# Autodesk Inventor assembly: Scrambler II
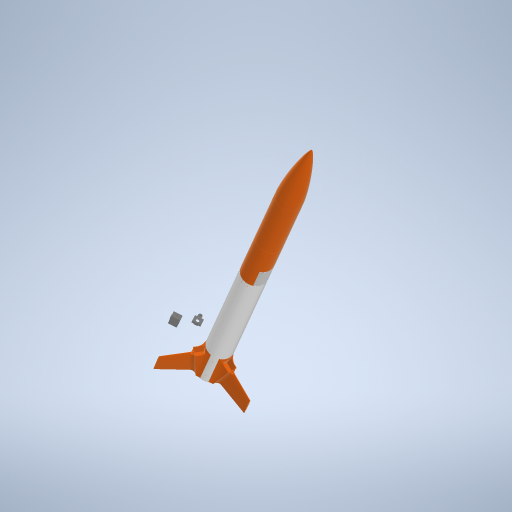
[picture p0: Inventor's stored thumbnail of the model, 512x512]
Saved by Autodesk Inventor 2024 (Build 280153000, 153)
## iProperties
Created: 2023-12-30
Part Number: Scrambler II
Document SubType Name: Assembly
Designer: Jamie
Mass: 631.455 g
Surface Area: 5625.65 cm^2
Volume: 391.502 cm^3
Density: 1.6129 g/cm^3
Author: Jamie
## Documents named in this file (10)
- C:\Users\auror\Documents\TU Delft\DARE\Git\Scrambler-2-CAD\Autodesk\Scrambler II.iam
- C:\Users\auror\Documents\TU Delft\DARE\Git\Scrambler-2-CAD\Autodesk\Structure.iam
- C:\Users\auror\Documents\TU Delft\DARE\Git\Scrambler-2-CAD\Autodesk\Lower skin.ipt
- C:\Users\auror\Documents\TU Delft\DARE\Git\Scrambler-2-CAD\Autodesk\Upper skin.ipt
- C:\Users\auror\Documents\TU Delft\DARE\Git\Scrambler-2-CAD\Autodesk\SRM with Smoke Grain.iam
- C:\Users\auror\Documents\TU Delft\DARE\Git\Scrambler-2-CAD\Autodesk\Nose assembly.iam
- C:\Users\auror\Documents\TU Delft\DARE\Git\Scrambler-2-CAD\Autodesk\Runcam.ipt
- C:\Users\auror\Documents\TU Delft\DARE\Git\Scrambler-2-CAD\Autodesk\Engine retention.ipt
- C:\Users\auror\Documents\TU Delft\DARE\Git\Scrambler-2-CAD\Autodesk\Electronic Assembly.iam
- C:\Users\auror\Documents\TU Delft\DARE\Git\Scrambler-2-CAD\Autodesk\Electronics Door.ipt
## Components (9 placed, 9 different names)
1. Structure:1 [sub-assembly] — Mate:1, Mate:2, Mate:3, Mate:4, Mate:30, Mate:31, Mate:32, Mate:33, Mate:34, Mate:35
2. Lower skin:1 — Mate:1, Mate:2, Mate:36, Mate:37, Mate:38, Mate:39
3. Upper skin:1 — Mate:3, Mate:4, Mate:9, Mate:10, Mate:11, Mate:29
4. SRM with Smoke Grain:1 [sub-assembly] — Mate:16, Mate:30, Mate:31
5. Nose assembly:1 [sub-assembly] — Mate:9, Mate:10, Mate:11, Mate:29
6. Runcam:1
7. Engine retention:1 — Mate:16, Mate:32
8. Electronic Assembly:1 [sub-assembly] — Mate:33, Mate:34, Mate:35
9. Electronics Door:1 — Mate:36, Mate:37, Mate:38, Mate:39
## Relationships (19: Mate 19)
- Mate:1: Structure:1 ↔ Lower skin:1
- Mate:2: Structure:1 ↔ Lower skin:1
- Mate:3: Structure:1 ↔ Upper skin:1
- Mate:4: Structure:1 ↔ Upper skin:1
- Mate:9: Upper skin:1 ↔ Nose assembly:1
- Mate:10: Upper skin:1 ↔ Nose assembly:1
- Mate:11: Upper skin:1 ↔ Nose assembly:1
- Mate:16: SRM with Smoke Grain:1 ↔ Engine retention:1
- Mate:29: Upper skin:1 ↔ Nose assembly:1
- Mate:30: Structure:1 ↔ SRM with Smoke Grain:1
- Mate:31: Structure:1 ↔ SRM with Smoke Grain:1
- Mate:32: Structure:1 ↔ Engine retention:1
- Mate:33: Structure:1 ↔ Electronic Assembly:1
- Mate:34: Structure:1 ↔ Electronic Assembly:1
- Mate:35: Structure:1 ↔ Electronic Assembly:1
- Mate:36: Lower skin:1 ↔ Electronics Door:1
- Mate:37: Lower skin:1 ↔ Electronics Door:1
- Mate:38: Lower skin:1 ↔ Electronics Door:1
- Mate:39: Lower skin:1 ↔ Electronics Door:1
